# Autodesk Inventor assembly: LIBSコリメータ
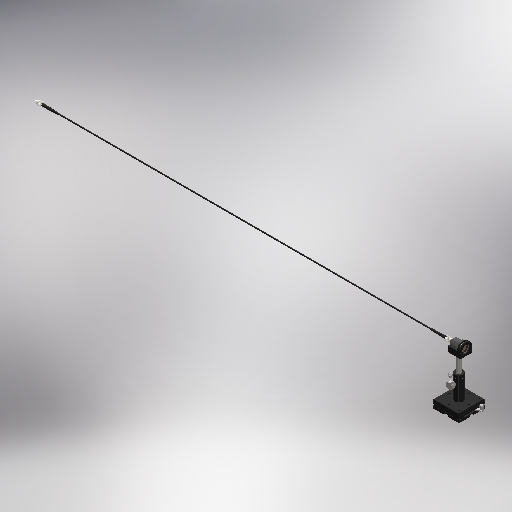
[picture p0: Inventor's stored thumbnail of the model, 512x512]
Saved by Autodesk Inventor 2026 (Build 300175050, 175E)
## iProperties
Created: 2025-08-17
Part Number: LIBSコリメータ
Document SubType Name: Assembly
Designer: jin20
Author: jin20
## Documents named in this file (4)
- C:\Users\jin20\Documents\装置CAD\SpectroscopySystem\Optics\LIBSコリメータ.iam
- C:\Users\jin20\Documents\装置CAD\SpectroscopySystem\Optics\コリメータ_エッジフィルター.iam
- C:\Users\jin20\Documents\装置CAD\SpectroscopySystem\Optics\光ファイバー.ipt
- C:\Users\jin20\Documents\装置CAD\SpectroscopySystem\Stage\マグネットベース.ipt
## Components (3 placed, 3 different names)
1. コリメータ_エッジフィルター:1 [sub-assembly] — 挿入:1, 挿入:2
2. 光ファイバー:1 — 挿入:2
3. マグネットベース:1 — 挿入:1
## Relationships (2: Insert 2)
- 挿入:1 [Insert]: コリメータ_エッジフィルター:1 ↔ マグネットベース:1
- 挿入:2 [Insert]: コリメータ_エッジフィルター:1 ↔ 光ファイバー:1
